# Autodesk Inventor assembly: KOGANEI_BDA10X15
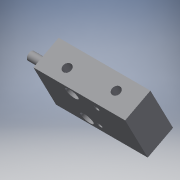
[picture p0: Inventor's stored thumbnail of the model, 180x180]
Saved by Autodesk Inventor 2018 (Build 220112000, 112)
## iProperties
Created: 2018-04-28
Part Number: KOGANEI_BDA10X15
Material: 一般
Document SubType Name: Assembly
Designer: Take
Author: Take
## Documents named in this file (3)
- C:\Users\Take\Documents\Inventor\パーツ\KOGANEI_BDA10X15.iam
- C:\Users\Take\Documents\Inventor\パーツ\KOGANEI_BDA10X15(円柱).ipt
- C:\Users\Take\Documents\Inventor\パーツ\KOGANEI_BDA10X15(本体).ipt
## Components (2 placed, 2 different names)
1. KOGANEI_BDA10X15(円柱):1 — 円柱状:1
2. KOGANEI_BDA10X15(本体):1 — 円柱状:1
## Relationships (1: CylindricalJoint 1)
- 円柱状:1 [CylindricalJoint]: KOGANEI_BDA10X15(円柱):1 ↔ KOGANEI_BDA10X15(本体):1
